# Autodesk Inventor assembly: PlanetaryGearbox
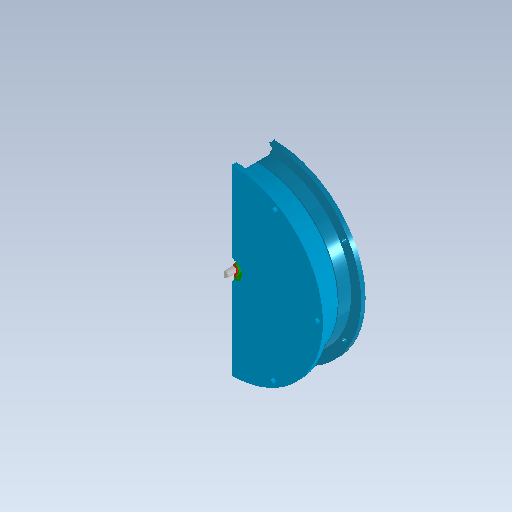
[picture p0: Inventor's stored thumbnail of the model, 512x512]
Saved by Autodesk Inventor 2021 (Build 250183000, 183)
## iProperties
Created: 2020-05-11
Part Number: PlanetaryGearbox
Document SubType Name: Assembly
Designer: avi41
Author: avi41
## Documents named in this file (14)
- C:\Users\avi41\Desktop\Robot Arm\CAD_files\PlanetaryGearbox_stage.iam
- C:\Users\avi41\Desktop\Robot Arm\CAD_files\Ring_gear.ipt
- C:\Users\avi41\Desktop\Robot Arm\CAD_files\Stage1_sun_gear.ipt
- C:\Users\avi41\Desktop\Robot Arm\CAD_files\Stage1_planet_gear.ipt
- C:\Users\avi41\Desktop\Robot Arm\CAD_files\Shaft_interstage.ipt
- C:\Users\avi41\Desktop\Robot Arm\CAD_files\Shaft_stage_input.ipt
- C:\Users\avi41\Desktop\Robot Arm\CAD_files\606.iam
- C:\Users\avi41\Desktop\Robot Arm\CAD_files\6-1287141.ipt
- C:\Users\avi41\Desktop\Robot Arm\CAD_files\Housing_stage.ipt
- C:\Users\avi41\Desktop\Robot Arm\CAD_files\HK0709FM.iam
- C:\Users\avi41\Desktop\Robot Arm\CAD_files\STWN7.ipt
- C:\Users\avi41\Desktop\Robot Arm\CAD_files\SC 0610CKP4.iam
- C:\Users\avi41\Documents\Inventor\Content Center Files\R2020\en-US\DIN 913\DIN 913 - M3 x 5.ipt
- C:\Users\avi41\Desktop\Robot Arm\CAD_files\Housing_stage_output.ipt
## Components (29 placed, 13 different names)
1. Ring_gear:1 — Mate:1, Mate:2, Flush:1, Mate:41, Flush:15, Flush:16, Flush:17, Flush:18, Mate:53
2. Stage1_planet_gear:1 — Mate:6, Mate:43, Flush:17, Mate:46, Mate:47, Mate:102
3. Stage1_planet_gear:2 — Mate:5, Flush:15, Mate:45, Mate:49
4. Stage1_planet_gear:3 — Mate:4, Flush:16, Mate:44, Mate:48
5. Shaft_interstage:1 — Mate:63, Mate:64, Mate:65, Mate:88, Flush:88, Mate:102
6. Shaft_stage_input:1 — Mate:39, Mate:40, Mate:54, Mate:56, Mate:57, Mate:58, Mate:59, Mate:60, Mate:61, Mate:82, Mate:83, Mate:84, Mate:85, Flush:87
7. 606:1 [sub-assembly] — Mate:42, Mate:52, Mate:54, Mate:62
8. 6-1287141:2 — Mate:39, Mate:40, Mate:62
9. Housing_stage:1 — Mate:41, Mate:42, Mate:52, Mate:53, Mate:92, Mate:93, Mate:101
10. HK0709FM:1 [sub-assembly] — Mate:44, Mate:48, Mate:63, Mate:64, Mate:69
11. HK0709FM:2 [sub-assembly] — Mate:43, Mate:46, Mate:47
12. HK0709FM:3 [sub-assembly] — Mate:45, Mate:49, Mate:68, Mate:70
13. Stage1_sun_gear:1 — Mate:51, Flush:18
14. 6-1287141:3 — Mate:56, Mate:57
15. 6-1287141:4 — Mate:58, Mate:59
16. 6-1287141:5 — Mate:60, Mate:61
17. STWN7:1 — Mate:70
18. STWN7:2 — Mate:68
19. STWN7:3 — Mate:65, Mate:69
20. 6-1287141:6 — Mate:89, Mate:103
21. 6-1287141:7 — Mate:90, Mate:91
22. SC 0610CKP4:1 [sub-assembly] — Mate:78, Mate:79, Mate:82, Mate:85, Flush:87
23. DIN 913 M3 x 5:1 — Mate:78, Mate:83, Mate:84
24. DIN 913 M3 x 5:2 — Mate:79
25. Shaft_stage_input:2 — Mate:88, Mate:89, Mate:90, Mate:91, Flush:88, Mate:96, Mate:98, Mate:103
26. Housing_stage_output:1 — Mate:92, Mate:93, Mate:94, Mate:95
27. 606:2 [sub-assembly] — Mate:94, Mate:95, Mate:97, Mate:99
28. 6-1287141:8 — Mate:96, Mate:97
29. 6-1287141:9 — Mate:98, Mate:99
## Relationships (61: Mate 54, Flush 7)
- Mate:1: Ring_gear:1
- Mate:2: Ring_gear:1
- Flush:1: Ring_gear:1
- Mate:4: Stage1_planet_gear:3
- Mate:5: Stage1_planet_gear:2
- Mate:6: Stage1_planet_gear:1
- Mate:39: Shaft_stage_input:1 ↔ 6-1287141:2
- Mate:40: Shaft_stage_input:1 ↔ 6-1287141:2
- Mate:41: Ring_gear:1 ↔ Housing_stage:1
- Mate:42: 606:1 ↔ Housing_stage:1
- Mate:43: Stage1_planet_gear:1 ↔ HK0709FM:2
- Flush:15: Ring_gear:1 ↔ Stage1_planet_gear:2
- Flush:16: Ring_gear:1 ↔ Stage1_planet_gear:3
- Flush:17: Ring_gear:1 ↔ Stage1_planet_gear:1
- Mate:44: Stage1_planet_gear:3 ↔ HK0709FM:1
- Mate:45: Stage1_planet_gear:2 ↔ HK0709FM:3
- Mate:46: Stage1_planet_gear:1 ↔ HK0709FM:2
- Mate:47: Stage1_planet_gear:1 ↔ HK0709FM:2
- Mate:48: Stage1_planet_gear:3 ↔ HK0709FM:1
- Mate:49: Stage1_planet_gear:2 ↔ HK0709FM:3
- Mate:51: Stage1_sun_gear:1
- Flush:18: Ring_gear:1 ↔ Stage1_sun_gear:1
- Mate:52: 606:1 ↔ Housing_stage:1
- Mate:53: Ring_gear:1 ↔ Housing_stage:1
- Mate:54: Shaft_stage_input:1 ↔ 606:1
- Mate:56: Shaft_stage_input:1 ↔ 6-1287141:3
- Mate:57: Shaft_stage_input:1 ↔ 6-1287141:3
- Mate:58: Shaft_stage_input:1 ↔ 6-1287141:4
- Mate:59: Shaft_stage_input:1 ↔ 6-1287141:4
- Mate:60: Shaft_stage_input:1 ↔ 6-1287141:5
- Mate:61: Shaft_stage_input:1 ↔ 6-1287141:5
- Mate:62: 606:1 ↔ 6-1287141:2
- Mate:63: Shaft_interstage:1 ↔ HK0709FM:1
- Mate:64: Shaft_interstage:1 ↔ HK0709FM:1
- Mate:65: Shaft_interstage:1 ↔ STWN7:3
- Mate:68: HK0709FM:3 ↔ STWN7:2
- Mate:69: HK0709FM:1 ↔ STWN7:3
- Mate:70: HK0709FM:3 ↔ STWN7:1
- Mate:78: SC 0610CKP4:1 ↔ DIN 913 M3 x 5:1
- Mate:79: SC 0610CKP4:1 ↔ DIN 913 M3 x 5:2
- Mate:82: Shaft_stage_input:1 ↔ SC 0610CKP4:1
- Mate:83 (3 mm): Shaft_stage_input:1 ↔ DIN 913 M3 x 5:1
- Mate:84 (3 mm): Shaft_stage_input:1 ↔ DIN 913 M3 x 5:1
- Mate:85: Shaft_stage_input:1 ↔ SC 0610CKP4:1
- Flush:87: Shaft_stage_input:1 ↔ SC 0610CKP4:1
- Mate:88: Shaft_interstage:1 ↔ Shaft_stage_input:2
- Mate:89: 6-1287141:6 ↔ Shaft_stage_input:2
- Mate:90: 6-1287141:7 ↔ Shaft_stage_input:2
- Mate:91: 6-1287141:7 ↔ Shaft_stage_input:2
- Flush:88: Shaft_interstage:1 ↔ Shaft_stage_input:2
- Mate:92: Housing_stage:1 ↔ Housing_stage_output:1
- Mate:93: Housing_stage:1 ↔ Housing_stage_output:1
- Mate:94: Housing_stage_output:1 ↔ 606:2
- Mate:95: Housing_stage_output:1 ↔ 606:2
- Mate:96: Shaft_stage_input:2 ↔ 6-1287141:8
- Mate:97: 606:2 ↔ 6-1287141:8
- Mate:98: Shaft_stage_input:2 ↔ 6-1287141:9
- Mate:99: 606:2 ↔ 6-1287141:9
- Mate:101: Housing_stage:1
- Mate:102: Stage1_planet_gear:1 ↔ Shaft_interstage:1
- Mate:103: 6-1287141:6 ↔ Shaft_stage_input:2
